# Autodesk Inventor assembly: Bibby Jordan Cody simple macine
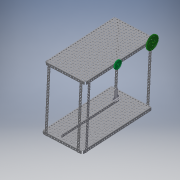
[picture p0: Inventor's stored thumbnail of the model, 180x180]
Saved by Autodesk Inventor 2018 (Build 220112000, 112)
## iProperties
Created: 2017-09-15
Part Number: Bibby Jordan Cody simple macine
Document SubType Name: Assembly
Designer: 196918
Author: 196918
## Documents named in this file (6)
- C:\Users\196918.FCBOE\Desktop\Bibby Jordan Cody simple macine.iam
- C:\Users\196918.FCBOE\Desktop\Vex Parts in Inventor\GEAR-60-TOOTH.ipt
- C:\Users\196918.FCBOE\Desktop\Vex Parts in Inventor\Angle-Gusset.ipt
- C:\Users\196918.FCBOE\Desktop\Vex Parts in Inventor\BAR 1X25 HOLES.ipt
- C:\Users\196918.FCBOE\Desktop\Vex Parts in Inventor\Base Plate.ipt
- C:\Users\196918.FCBOE\Desktop\Vex Parts in Inventor\GEAR-36-TOOTH.ipt
## Components (11 placed, 5 different names)
1. GEAR-60-TOOTH:1 — Rigid:7
2. Angle-Gusset:1 — Flush:3, Flush:4, Flush:5
3. BAR 1X25 HOLES:1 — Rigid:5, Rigid:6
4. Base Plate:1 — Mate:1, Flush:1, Flush:2, Rigid:7, Rigid:8
5. Base Plate:2 — Rigid:1, Rigid:2, Rigid:3, Rigid:4, Rigid:5
6. BAR 1X25 HOLES:2 — Rigid:1, Flush:1, Flush:2
7. BAR 1X25 HOLES:3 — Rigid:2
8. BAR 1X25 HOLES:4 — Rigid:3
9. BAR 1X25 HOLES:5 — Rigid:4, Mate:1
10. BAR 1X25 HOLES:6 — Rigid:6, Flush:3, Flush:4, Flush:5
11. GEAR-36-TOOTH:1 — Rigid:8
## Relationships (14: WeldJoint 8, Flush 5, Mate 1)
- Rigid:1 [WeldJoint]: Base Plate:2 ↔ BAR 1X25 HOLES:2
- Rigid:2 [WeldJoint]: Base Plate:2 ↔ BAR 1X25 HOLES:3
- Rigid:3 [WeldJoint]: Base Plate:2 ↔ BAR 1X25 HOLES:4
- Rigid:4 [WeldJoint]: Base Plate:2 ↔ BAR 1X25 HOLES:5
- Mate:1: Base Plate:1 ↔ BAR 1X25 HOLES:5
- Flush:1: Base Plate:1 ↔ BAR 1X25 HOLES:2
- Flush:2: Base Plate:1 ↔ BAR 1X25 HOLES:2
- Rigid:5 [WeldJoint]: BAR 1X25 HOLES:1 ↔ Base Plate:2
- Rigid:6 [WeldJoint]: BAR 1X25 HOLES:1 ↔ BAR 1X25 HOLES:6
- Rigid:7 [WeldJoint]: GEAR-60-TOOTH:1 ↔ Base Plate:1
- Rigid:8 [WeldJoint]: Base Plate:1 ↔ GEAR-36-TOOTH:1
- Flush:3: Angle-Gusset:1 ↔ BAR 1X25 HOLES:6
- Flush:4: Angle-Gusset:1 ↔ BAR 1X25 HOLES:6
- Flush:5 (-50.8 mm): Angle-Gusset:1 ↔ BAR 1X25 HOLES:6
